# Autodesk Inventor assembly: sampleHolderAssembly
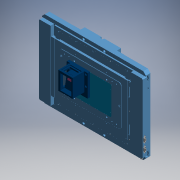
[picture p0: Inventor's stored thumbnail of the model, 180x180]
Saved by Autodesk Inventor 2016 (Build 200138000, 138)
## iProperties
Created: 2016-04-09
Part Number: sampleHolderAssembly
Document SubType Name: Assembly
Designer: sims01
Author: sims01
## Documents named in this file (5)
- H:\Documents\LSFM_3\setup\mechanical\design\lsfm3_mechDesign\sampleHolderAssembly.iam
- H:\Documents\LSFM_3\setup\mechanical\design\lsfm3_mechDesign\piStage_XY.ipt
- H:\Documents\LSFM_3\setup\mechanical\design\lsfm3_mechDesign\sampleHolderBase.ipt
- H:\Documents\LSFM_3\setup\mechanical\design\lsfm3_mechDesign\filipeTestSample.ipt
- H:\Documents\LSFM_3\setup\mechanical\design\lsfm3_mechDesign\sampleChamber_singlePiece_filipeSample.ipt
## Components (4 placed, 4 different names)
1. piStage_XY:1 — Rigid:4
2. filipeTestSample:1 — Rigid:3
3. sampleChamber_singlePiece_filipeSample:1 — Rigid:3, Rigid:5
4. sampleHolderBase:1 — Rigid:4, Rigid:5
## Relationships (3: WeldJoint 3)
- Rigid:3 [WeldJoint]: filipeTestSample:1 ↔ sampleChamber_singlePiece_filipeSample:1
- Rigid:4 [WeldJoint]: piStage_XY:1 ↔ sampleHolderBase:1
- Rigid:5 [WeldJoint]: sampleChamber_singlePiece_filipeSample:1 ↔ sampleHolderBase:1
